# Autodesk Inventor assembly: wheelchair_sm_varx
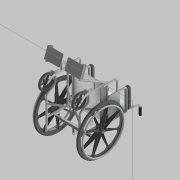
[picture p0: Inventor's stored thumbnail of the model, 180x180]
Saved by Autodesk Inventor 2021 (Build 250183000, 183)
## iProperties
Created: 2021-06-02
Part Number: wheelchair_sm_varx
Document SubType Name: Assembly
Designer: Watchdog
Author: Watchdog
## Documents named in this file (3)
- C:\Users\Watchdog\OneDrive - Flinders\Advn Mech Design Shared\6_Development\2_Design\inventor\vehicle_wheelchair\wheelchair\wheelchair_sm_varx.iam
- C:\Users\Watchdog\OneDrive - Flinders\Advn Mech Design Shared\6_Development\2_Design\inventor\vehicle_wheelchair\wheelchair\wheelchair_hypoth.ipt
- C:\Users\Watchdog\OneDrive - Flinders\Advn Mech Design Shared\6_Development\2_Design\inventor\securing_mechanism\securingMechanism_variant_vertical_x\sm_varx.iam
## Components (2 placed, 2 different names)
1. wheelchair_hypoth:1 — Flush:1, Mate:1, Mate:2, Mate:3, Flush:2, Flush:3
2. sm_varx:1 [sub-assembly] — Mate:3, Flush:2, Flush:3
## Relationships (6: Flush 3, Mate 3)
- Flush:1: wheelchair_hypoth:1
- Mate:1: wheelchair_hypoth:1
- Mate:2: wheelchair_hypoth:1
- Mate:3: wheelchair_hypoth:1 ↔ sm_varx:1
- Flush:2: wheelchair_hypoth:1 ↔ sm_varx:1
- Flush:3: wheelchair_hypoth:1 ↔ sm_varx:1
